# Autodesk Inventor assembly: BeltDrive
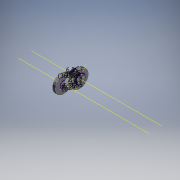
[picture p0: Inventor's stored thumbnail of the model, 180x180]
Saved by Autodesk Inventor 2018.3 (Build 223284000, 284)
## iProperties
Created: 2018-07-29
Part Number: BeltDrive
Material: Generisch
Document SubType Name: Assembly
Designer: JochenAlt
Author: JochenAlt
## Documents named in this file (4)
- D:\Projects\FlowerPot\CAD\Beltdrive\BeltDrive.iam
- D:\Projects\FlowerPot\CAD\Beltdrive\BeltDriveConstruction.iam
- D:\Projects\FlowerPot\CAD\Mounting Hub.ipt
- D:\Projects\FlowerPot\CAD\Beltdrive\ZwischenScheiben.ipt
## Components (4 placed, 3 different names)
1. BeltDriveConstruction:1 [sub-assembly] — Passend:5, Passend:6, Passend:13, Passend:15, Drehung:2, Passend:16, Passend:17, Passend:18, Passend:20, Passend:21, Passend:22
2. Mounting Hub:1 — Passend:5, Passend:6
3. Synchrone Riemenscheibe1:1 — Passend:13, Drehung:2, Passend:17, Passend:22
4. Mounting Hub:2 — Passend:19, Passend:20, Passend:21
## Relationships (12: Mate 11, RelateRotation 1)
- Passend:5 [Mate]: BeltDriveConstruction:1 ↔ Mounting Hub:1
- Passend:6 [Mate]: BeltDriveConstruction:1 ↔ Mounting Hub:1
- Passend:13 [Mate]: BeltDriveConstruction:1 ↔ Synchrone Riemenscheibe1:1
- Passend:15 [Mate]: BeltDriveConstruction:1
- Drehung:2 [RelateRotation] (0.3333 ul): BeltDriveConstruction:1 ↔ Synchrone Riemenscheibe1:1
- Passend:16 [Mate]: BeltDriveConstruction:1
- Passend:17 [Mate] (1 mm): BeltDriveConstruction:1 ↔ Synchrone Riemenscheibe1:1
- Passend:18 [Mate]: BeltDriveConstruction:1
- Passend:19 [Mate]: Mounting Hub:2
- Passend:20 [Mate]: BeltDriveConstruction:1 ↔ Mounting Hub:2
- Passend:21 [Mate]: BeltDriveConstruction:1 ↔ Mounting Hub:2
- Passend:22 [Mate]: BeltDriveConstruction:1 ↔ Synchrone Riemenscheibe1:1
